# Autodesk Inventor assembly: MJT-30-BL-8-12
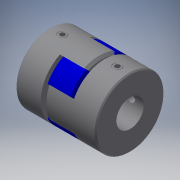
[picture p0: Inventor's stored thumbnail of the model, 180x180]
Saved by Autodesk Inventor 2019 (Build 230136000, 136)
## iProperties
Category: PARTsolutions
Company: NBK
Created: 2023-09-29
Part Number: MJT-30-BL-8-12
Catalog Web Link: www.cadenas.de
Description: MJT-
Vendor: NBK
Document SubType Name: Assembly
Designer: psAdmin
Manufacturer: NBK
Mass: 20.9954 g
Surface Area: 90.0424 cm^2
Volume: 20.9954 cm^3
Density: 1 g/cm^3
Title: MJT-30-BL-8-12
Author: Cadenas PARTsolutions
PSOL_IDENT_0: {$CADENAS_DATA/23d-libs/nbk/motion_control_parts/couplicon_mini/jaw_type/mjt/mjt_asmtab.prj},184 {VT
PSOL_IDENT_1: YP=3D},{STYP=ASSTAB},{NB=MJT-30-BL-8-12},{LINA=MJT-30-BL-8-12},{NN=MJT},{DATE=25.09.2023 00:41:45},{
PSOL_IDENT_2: GEOMDATE=12.03.2020 14:00:36},{VERSION=},{LINEID=200},{WBVAR=D1D2},{WBNUMERIC=}  {NB=MJT-30-BL-8-12}
PSOL_IDENT_3: ,{LINA=MJT-30-BL-8-12},{KT=DUMMY},{CN=MJT-30-BL},{D1D2=8-12},{D1D2X1='6-6','6-6.35','6-7','6-8','6-9
PSOL_IDENT_4: .525','6-10','6-11','6-12','6-14','6-15','6-16','6.35-6.35','6.35-7','6.35-8','6.35-9.525','6.35-10'
PSOL_IDENT_5: ,'6.35-11','6.35-12','6.35-14','6.35-15','6.35-16','7-7','7-8','7-9.525','7-10','7-11','7-12','7-14'
PSOL_IDENT_6: ,'7-15','7-16','8-8','8-9.525','8-10','8-11','8-12','8-14','8-15','8-16','9.525-9.525','9.525-10','9
PSOL_IDENT_7: .525-11','9.525-12','9.525-14','9.525-15','9.525-16','10-10','10-11','10-12','10-14','10-15','10-16'
PSOL_IDENT_8: ,'11-11','11-12','11-14','11-15','11-16','12-12','12-14','12-15','12-16','14-14','14-15','14-16','15
PSOL_IDENT_9: -15','15-16','16-16'},{A=30},{L=11},{W=35},{B=10},{C=1.5},{F=5.5},{M=M4},{WT=1.7},{D1=8},{D2=12},{PP
PSOL_IDENT_10: ATH=mjt_asmtpl.prj},{KV=0},{CNSORDERNO=MJT-30-BL-8-12}
NB: MJT-30-BL-8-12
NN: MJT
NBSYN: $CNSORDERNO.
LINA: MJT-30-BL-8-12
CATALOG: NBK (Nabeya Bi-tech Kaisha
CN: MJT-30-BL
D1D2: 8-12
A: 30
L: 11
W: 35
B: 10
C: 1.5
F: 5.5
M: M4
WT: 1.7
SUPPLIER: NBK
ARTICLENO: MJT-30-BL-8-12
BOMINFO: MJT-30-BL-8-12
CREATOR: CADENAS GmbH
## Documents named in this file (4)
- e:\temp\worker_COMMON_2\temp\tmp_2080_196_tmt8n\format_0\MJT-30-BL-8-12.iam
- e:\temp\worker_COMMON_2\temp\tmp_2080_196_tmt8n\format_0\MJT-30-BL-8-12 Hub 1.ipt
- e:\temp\worker_COMMON_2\temp\tmp_2080_196_tmt8n\format_0\MJT-30-BL Sleeve.ipt
- e:\temp\worker_COMMON_2\temp\tmp_2080_196_tmt8n\format_0\MJT-30-BL-8-12 Hub 2.ipt
## Components (3 placed, 3 different names)
1. MJT-30-BL-8-12 Hub 1:1 — part1b_XY@1 <-> part2a_XY@2, part1b_Z@1 <-> part2a_Z@2, part1b_YZ@1 <-> part2a_YZ@2, part1c_XY@1 <-> part3_XY@3, part1c_Z@1 <-> part3_Z@3, part1c_YZ@1 <-> part3_YZ@3
2. MJT-30-BL Sleeve:1 — part1b_XY@1 <-> part2a_XY@2, part1b_Z@1 <-> part2a_Z@2, part1b_YZ@1 <-> part2a_YZ@2
3. MJT-30-BL-8-12 Hub 2:1 — part1c_XY@1 <-> part3_XY@3, part1c_Z@1 <-> part3_Z@3, part1c_YZ@1 <-> part3_YZ@3
## Relationships (6: Flush 2, Mate 2, Angle 2)
- part1b_XY@1 <-> part2a_XY@2 [Flush]: MJT-30-BL-8-12 Hub 1:1 ↔ MJT-30-BL Sleeve:1
- part1b_Z@1 <-> part2a_Z@2 [Mate]: MJT-30-BL-8-12 Hub 1:1 ↔ MJT-30-BL Sleeve:1
- part1b_YZ@1 <-> part2a_YZ@2 [Angle] (0 deg): MJT-30-BL-8-12 Hub 1:1 ↔ MJT-30-BL Sleeve:1
- part1c_XY@1 <-> part3_XY@3 [Flush]: MJT-30-BL-8-12 Hub 1:1 ↔ MJT-30-BL-8-12 Hub 2:1
- part1c_Z@1 <-> part3_Z@3 [Mate]: MJT-30-BL-8-12 Hub 1:1 ↔ MJT-30-BL-8-12 Hub 2:1
- part1c_YZ@1 <-> part3_YZ@3 [Angle] (0 deg): MJT-30-BL-8-12 Hub 1:1 ↔ MJT-30-BL-8-12 Hub 2:1
